# Autodesk Inventor assembly: WheelNGearmk2
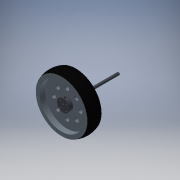
[picture p0: Inventor's stored thumbnail of the model, 180x180]
Saved by Autodesk Inventor 2016 (Build 200138000, 138)
## iProperties
Created: 2015-08-30
Part Number: WheelNGearmk2
Document SubType Name: Assembly
Designer: Tim
Author: Tim
## Documents named in this file (6)
- C:\Users\phi\Documents\GitHub\phi_robotics\3d-models\FTC_Tetrix_KOP_Block_Party\Tim Bloot Designs\WheelNGearmk2.iam
- C:\Users\phi\Documents\GitHub\phi_robotics\3d-models\FTC_Tetrix_KOP_Block_Party\Tetrix_Kit_FTC\Autodesk Inventor Files\tetrix_wheel.ipt
- C:\Users\phi\Documents\GitHub\phi_robotics\3d-models\FTC_Tetrix_KOP_Block_Party\Tetrix_Kit_FTC\Autodesk Inventor Files\tetrix_gear-med.ipt
- C:\Users\phi\Documents\GitHub\phi_robotics\3d-models\FTC_Tetrix_KOP_Block_Party\Tetrix_Kit_FTC\Autodesk Inventor Files\tetrix_axle_lock.iam
- C:\Users\phi\Documents\GitHub\phi_robotics\3d-models\FTC_Tetrix_KOP_Block_Party\Tetrix_Kit_FTC\Autodesk Inventor Files\tetrix_axle_spacer_mount.ipt
- C:\Users\phi\Documents\GitHub\phi_robotics\3d-models\FTC_Tetrix_KOP_Block_Party\Tetrix_Kit_FTC\Autodesk Inventor Files\tetrix_axle.ipt
## Components (6 placed, 5 different names)
1. tetrix_wheel:1 — Rigid:1, Rigid:4
2. tetrix_gear-med:1 — Rigid:2, Rigid:3
3. tetrix_axle_lock:1 [sub-assembly] — Rigid:4, Rigid:5
4. tetrix_axle_lock:2 [sub-assembly] — Rigid:3
5. tetrix_axle_spacer_mount:1 — Rigid:1, Rigid:2
6. tetrix_axle:1 — Rigid:5
## Relationships (5: WeldJoint 5)
- Rigid:1 [WeldJoint]: tetrix_wheel:1 ↔ tetrix_axle_spacer_mount:1
- Rigid:2 [WeldJoint]: tetrix_gear-med:1 ↔ tetrix_axle_spacer_mount:1
- Rigid:3 [WeldJoint]: tetrix_gear-med:1 ↔ tetrix_axle_lock:2
- Rigid:4 [WeldJoint]: tetrix_wheel:1 ↔ tetrix_axle_lock:1
- Rigid:5 [WeldJoint] (-1 mm): tetrix_axle_lock:1 ↔ tetrix_axle:1
